# Autodesk Inventor assembly: A2017_T4_01
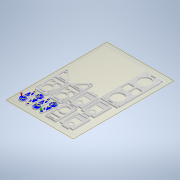
[picture p0: Inventor's stored thumbnail of the model, 180x180]
Saved by Autodesk Inventor 2020 (Build 240168000, 168)
## iProperties
Created: 2021-08-27
Part Number: A2017_T4_01
Document SubType Name: Assembly
Designer: Masato
Author: Masato
## Documents named in this file (8)
- C:\Users\marin\Documents\0228 git clone\OpenPlatform_ver3_0\Cam\A2017_T4_01.iam
- C:\Users\marin\Documents\0228 git clone\OpenPlatform_ver3_0\Cam\DisposableBoard.ipt
- C:\Users\marin\Documents\0228 git clone\OpenPlatform_ver3_0\LowerBody\Ankle\Ankle_side_pitch_frame.ipt
- C:\Users\marin\Documents\0228 git clone\OpenPlatform_ver3_0\UpperBody\Trunk\Trunk_neck_frame.ipt
- C:\Users\marin\Documents\0228 git clone\OpenPlatform_ver3_0\UpperBody\Trunk\Trunk_shoulder_frame.ipt
- C:\Users\marin\Documents\0228 git clone\OpenPlatform_ver3_0\UpperBody\Trunk\Trunk_shoulder_frame_MIR.ipt
- C:\Users\marin\Documents\0228 git clone\OpenPlatform_ver3_0\UpperBody\Trunk\Trunk_waisit_frame.ipt
- C:\Users\marin\Documents\0228 git clone\OpenPlatform_ver3_0\UpperBody\Trunk\Trunk_servo_bottom_frame.ipt
## Components (12 placed, 7 different names)
1. DisposableBoard:1 — メイト:2, メイト:1, フラッシュ:1, フラッシュ:2, 角度:1, 正接:1, 正接:2, 角度:2, 正接:3, フラッシュ:3, フラッシュ:5, フラッシュ:6, フラッシュ:7
2. Trunk_neck_frame:1 — メイト:6, フラッシュ:3, 正接:6, メイト:13, メイト:15
3. Trunk_shoulder_frame:1 — メイト:9, フラッシュ:5, メイト:11, 正接:7
4. Trunk_shoulder_frame_MIR:1 — メイト:10, メイト:11, 正接:8, メイト:16
5. Trunk_waisit_frame:1 — メイト:7, メイト:17, フラッシュ:7
6. Trunk_servo_bottom_frame:2 — メイト:14, メイト:15, メイト:16
7. Ankle_side_pitch_frame:1 — メイト:4, 角度:1, 正接:1, 正接:2, 正接:4
8. Ankle_side_pitch_frame:2 — メイト:5, 角度:2, 正接:3, 正接:4, 正接:7
9. Ankle_side_pitch_frame:3
10. Ankle_side_pitch_frame:4 — 正接:6, 正接:8
11. Trunk_servo_bottom_frame:1 — メイト:12, フラッシュ:6, メイト:13
12. Trunk_servo_bottom_frame:3 — メイト:17
## Component patterns: (2 elements, first: Ankle_side_pitch_frame:1 + Ankle_side_pitch_frame:2), (2 elements, first: Trunk_servo_bottom_frame:1)
## Relationships (30: Mate 15, Tangent 7, Flush 6, Angle 2)
- メイト:2 [Mate]: DisposableBoard:1
- メイト:1 [Mate]: DisposableBoard:1
- フラッシュ:1 [Flush]: DisposableBoard:1
- フラッシュ:2 [Flush]: DisposableBoard:1
- メイト:4 [Mate]: Ankle_side_pitch_frame:1
- 角度:1 [Angle] (0 deg): DisposableBoard:1 ↔ Ankle_side_pitch_frame:1
- 正接:1 [Tangent] (3 mm): DisposableBoard:1 ↔ Ankle_side_pitch_frame:1
- 正接:2 [Tangent] (3 mm): DisposableBoard:1 ↔ Ankle_side_pitch_frame:1
- メイト:5 [Mate]: Ankle_side_pitch_frame:2
- 角度:2 [Angle] (0 deg): DisposableBoard:1 ↔ Ankle_side_pitch_frame:2
- 正接:3 [Tangent] (3 mm): DisposableBoard:1 ↔ Ankle_side_pitch_frame:2
- 正接:4 [Tangent] (2.5 mm): Ankle_side_pitch_frame:1 ↔ Ankle_side_pitch_frame:2
- メイト:6 [Mate]: Trunk_neck_frame:1
- フラッシュ:3 [Flush] (3 mm): DisposableBoard:1 ↔ Trunk_neck_frame:1
- メイト:7 [Mate]: Trunk_waisit_frame:1
- メイト:9 [Mate]: Trunk_shoulder_frame:1
- フラッシュ:5 [Flush] (3 mm): DisposableBoard:1 ↔ Trunk_shoulder_frame:1
- メイト:10 [Mate]: Trunk_shoulder_frame_MIR:1
- メイト:11 [Mate] (2.5 mm): Trunk_shoulder_frame:1 ↔ Trunk_shoulder_frame_MIR:1
- 正接:6 [Tangent] (2.5 mm): Trunk_neck_frame:1 ↔ Ankle_side_pitch_frame:4
- 正接:7 [Tangent] (2.5 mm): Trunk_shoulder_frame:1 ↔ Ankle_side_pitch_frame:2
- 正接:8 [Tangent] (2.5 mm): Trunk_shoulder_frame_MIR:1 ↔ Ankle_side_pitch_frame:4
- メイト:12 [Mate]: Trunk_servo_bottom_frame:1
- フラッシュ:6 [Flush] (3 mm): DisposableBoard:1 ↔ Trunk_servo_bottom_frame:1
- メイト:13 [Mate] (6.6 mm): Trunk_neck_frame:1 ↔ Trunk_servo_bottom_frame:1
- メイト:14 [Mate]: Trunk_servo_bottom_frame:2
- メイト:15 [Mate] (2.5 mm): Trunk_neck_frame:1 ↔ Trunk_servo_bottom_frame:2
- メイト:16 [Mate] (2.5 mm): Trunk_shoulder_frame_MIR:1 ↔ Trunk_servo_bottom_frame:2
- メイト:17 [Mate] (2.5 mm): Trunk_waisit_frame:1 ↔ Trunk_servo_bottom_frame:3
- フラッシュ:7 [Flush] (3 mm): DisposableBoard:1 ↔ Trunk_waisit_frame:1
